# Autodesk Inventor assembly: UR5Assem
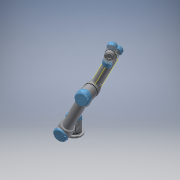
[picture p0: Inventor's stored thumbnail of the model, 180x180]
Saved by Autodesk Inventor 2018 (Build 220112000, 112)
## iProperties
Created: 2019-04-06
Part Number: UR5Assem
Description: STEP AP214
Document SubType Name: Assembly
Designer: Jesse R-B
Sending System: SolidWorks 2019
Preprocessor: SwSTEP 2.0
Title: UR5.STEP
Revision Number: ANY
## Documents named in this file (8)
- C:\Users\Jesse R-B\Documents\Inventor\400\ur5-5.snapshot.3\UR5Assem.iam
- C:\Users\Jesse R-B\Documents\Inventor\400\ur5-5.snapshot.3\Base.iam
- C:\Users\Jesse R-B\Documents\Inventor\400\ur5-5.snapshot.3\J1.iam
- C:\Users\Jesse R-B\Documents\Inventor\400\ur5-5.snapshot.3\J2.iam
- C:\Users\Jesse R-B\Documents\Inventor\400\ur5-5.snapshot.3\J3.iam
- C:\Users\Jesse R-B\Documents\Inventor\400\ur5-5.snapshot.3\J4.iam
- C:\Users\Jesse R-B\Documents\Inventor\400\ur5-5.snapshot.3\J5.iam
- C:\Users\Jesse R-B\Documents\Inventor\400\ur5-5.snapshot.3\J6.iam
## Components (7 placed, 7 different names)
1. Base_1 [sub-assembly] — Mate:11, Mate:12
2. J1_2 [sub-assembly] — Mate:9, Mate:10, Mate:11, Mate:12
3. J2_3 [sub-assembly] — Mate:7, Mate:8, Mate:9, Mate:10
4. J3_4 [sub-assembly] — Mate:5, Mate:6, Mate:7, Mate:8
5. J4_5 [sub-assembly] — Mate:3, Mate:4, Mate:5, Mate:6
6. J5_6 [sub-assembly] — Mate:1, Mate:2, Mate:3, Mate:4
7. J6_7 [sub-assembly] — Mate:1, Mate:2
## Relationships (12: Mate 12)
- Mate:1: J5_6 ↔ J6_7
- Mate:2: J5_6 ↔ J6_7
- Mate:3: J4_5 ↔ J5_6
- Mate:4: J4_5 ↔ J5_6
- Mate:5: J3_4 ↔ J4_5
- Mate:6: J3_4 ↔ J4_5
- Mate:7: J2_3 ↔ J3_4
- Mate:8: J2_3 ↔ J3_4
- Mate:9: J1_2 ↔ J2_3
- Mate:10: J1_2 ↔ J2_3
- Mate:11: Base_1 ↔ J1_2
- Mate:12: Base_1 ↔ J1_2
